# Autodesk Inventor assembly: Montagem Morsa Vista Explodida
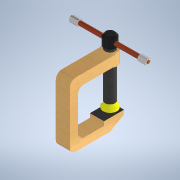
[picture p0: Inventor's stored thumbnail of the model, 180x180]
Saved by Autodesk Inventor 2021 (Build 250183000, 183)
## iProperties
Created: 2021-05-13
Part Number: Montagem Morsa Vista Explodida
Document SubType Name: Assembly
Designer: rubia
Author: rubia
## Documents named in this file (6)
- C:\Users\rubia\OneDrive\Documentos\Inventor\Rubia_ASR9\Montagem Morsa Vista Explodida.iam
- C:\Users\rubia\OneDrive\Documentos\Inventor\Rubia_ASR9\Apoio da Haste.ipt
- C:\Users\rubia\OneDrive\Documentos\Inventor\Rubia_ASR9\Apoio da Morsa.ipt
- C:\Users\rubia\OneDrive\Documentos\Inventor\Rubia_ASR9\Corpo da Morsa.ipt
- C:\Users\rubia\OneDrive\Documentos\Inventor\Rubia_ASR9\Haste da Morsa.ipt
- C:\Users\rubia\OneDrive\Documentos\Inventor\Rubia_ASR9\Prisioneiro.ipt
## Components (6 placed, 5 different names)
1. Apoio da Haste:1 — Coincidente:9, Coincidente:10
2. Apoio da Morsa:1 — Coincidente:2, Coincidente:3, Coincidente:4
3. Corpo da Morsa:1 — Coincidente:1, Coincidente:4
4. Haste da Morsa:1 — Coincidente:9, Coincidente:10, Coincidente:11, Coincidente:12, Coincidente:13, Coincidente:14
5. Prisioneiro:1 — Coincidente:1, Coincidente:2, Coincidente:3, Coincidente:11, Coincidente:12
6. Apoio da Haste:2 — Coincidente:13, Coincidente:14
## Relationships (10: Mate 10)
- Coincidente:1 [Mate]: Corpo da Morsa:1 ↔ Prisioneiro:1
- Coincidente:2 [Mate]: Apoio da Morsa:1 ↔ Prisioneiro:1
- Coincidente:3 [Mate]: Apoio da Morsa:1 ↔ Prisioneiro:1
- Coincidente:4 [Mate] (10 mm): Apoio da Morsa:1 ↔ Corpo da Morsa:1
- Coincidente:9 [Mate]: Apoio da Haste:1 ↔ Haste da Morsa:1
- Coincidente:10 [Mate]: Apoio da Haste:1 ↔ Haste da Morsa:1
- Coincidente:11 [Mate]: Haste da Morsa:1 ↔ Prisioneiro:1
- Coincidente:12 [Mate] (-150 mm): Haste da Morsa:1 ↔ Prisioneiro:1
- Coincidente:13 [Mate]: Haste da Morsa:1 ↔ Apoio da Haste:2
- Coincidente:14 [Mate]: Haste da Morsa:1 ↔ Apoio da Haste:2
